# Autodesk Inventor assembly: test-side
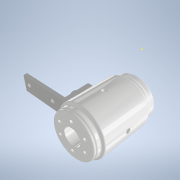
[picture p0: Inventor's stored thumbnail of the model, 180x180]
Saved by Autodesk Inventor 2020.1 (Build 241239000, 239)
## iProperties
Created: 2019-11-06
Part Number: test-side
Document SubType Name: Assembly
Designer: njk024
Author: njk024
## Documents named in this file (4)
- K:\OneDrive\Projects\Smart-Water-Quality-Sensor\Smart-Water-Quality-Sensor\mechanical\design\test-side.iam
- K:\OneDrive\Projects\Smart-Water-Quality-Sensor\Smart-Water-Quality-Sensor\mechanical\design\inside.ipt
- K:\OneDrive\Projects\Smart-Water-Quality-Sensor\Smart-Water-Quality-Sensor\mechanical\design\side-mounts-for-floater.ipt
- K:\OneDrive\Projects\Smart-Water-Quality-Sensor\Smart-Water-Quality-Sensor\mechanical\design\inside-mount.ipt
## Components (3 placed, 3 different names)
1. inside:1 — Mate:1, Mate:3, Mate:4
2. side-mounts-for-floater:1 — Mate:1
3. inside-mount:1 — Mate:3, Mate:4
## Relationships (3: Mate 3)
- Mate:1: inside:1 ↔ side-mounts-for-floater:1
- Mate:3: inside:1 ↔ inside-mount:1
- Mate:4: inside:1 ↔ inside-mount:1
